# Autodesk Inventor assembly: Final AssemblyV6
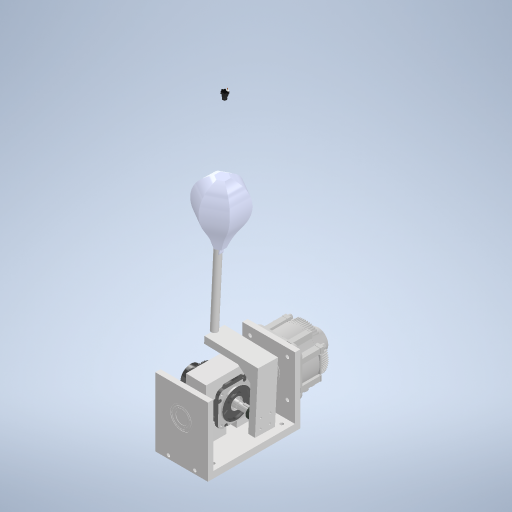
[picture p0: Inventor's stored thumbnail of the model, 512x512]
Saved by Autodesk Inventor 2024 (Build 280153000, 153)
## iProperties
Created: 2024-03-22
Part Number: Final AssemblyV6
Document SubType Name: Assembly
Designer: yusuf
Author: yusuf
## Documents named in this file (16)
- C:\Users\yusuf\Documents\DodgeBot\design\hardware\CAD_FILES\Final AssemblyV6.iam
- C:\Users\yusuf\Documents\DodgeBot\design\hardware\CAD_FILES\FloorMount.ipt
- C:\Users\yusuf\Documents\DodgeBot\design\hardware\CAD_FILES\145100992-9-skf_bearing_6209-2z_2\skf_bearing_6209-2z_2.iam
- C:\Users\yusuf\Documents\DodgeBot\design\hardware\CAD_FILES\FloorMountV2.ipt
- C:\Users\yusuf\Documents\DodgeBot\design\hardware\CAD_FILES\FloorMountFacePlate.ipt
- C:\Users\yusuf\Documents\DodgeBot\design\hardware\CAD_FILES\YASKAWA_USA_SGM7G30A6A61\AIS2024\SGM7G-30A6A61.iam
- C:\Users\yusuf\Documents\DodgeBot\design\hardware\CAD_FILES\grainger-big\grainger-big.iam
- C:\Users\yusuf\Documents\DodgeBot\design\hardware\CAD_FILES\FrontPlatePostNoKey.ipt
- C:\Users\yusuf\Documents\DodgeBot\design\hardware\CAD_FILES\EndEffector.ipt
- C:\Users\yusuf\Documents\DodgeBot\design\hardware\CAD_FILES\Speedbag\Speedbag.ipt
- C:\Users\yusuf\Documents\DodgeBot\design\hardware\CAD_FILES\grainger-small\grainger-small.iam
- C:\Users\yusuf\Documents\DodgeBot\design\hardware\CAD_FILES\SGM7G_20AxA61\SGM7G-20xxA61\ProE\SGM7G-20__a61_ProE\ProE\sgm7g_20__a61\sgm7g_20__a61.iam
- C:\Users\yusuf\Documents\DodgeBot\design\hardware\CAD_FILES\Post.ipt
- C:\Users\yusuf\Documents\DodgeBot\design\hardware\CAD_FILES\FrontPlatePostEndSide.ipt
- C:\Users\yusuf\Documents\DodgeBot\design\hardware\CAD_FILES\FrontPlateV3.ipt
- C:\Users\yusuf\Documents\DodgeBot\design\hardware\CAD_FILES\1000TVL v6\1000TVL v6.ipt
## Components (16 placed, 15 different names)
1. FloorMountV2:1 — Rigid:1, Rigid:2
2. FloorMountFacePlate:2 — Rigid:1, Rotational:1
3. skf_bearing_6209-2z_2:1 [sub-assembly] — Rotational:1, Rotational:10
4. skf_bearing_6209-2z_2:2 [sub-assembly] — Rotational:2
5. SGM7G-30A6A61:1 [sub-assembly] — Rigid:3, Rigid:10
6. FloorMount:1 — Rigid:2, Rotational:2, Rigid:3
7. grainger-big:1 [sub-assembly] — Rigid:10
8. EndEffector:1 — Rigid:7, Rotational:16, Rigid:15
9. Speedbag:1 — Rigid:6
10. grainger-small:1 [sub-assembly] — Rigid:12, Rotational:16
11. sgm7g_20__a61:1 [sub-assembly] — Rigid:12, Rotational:11
12. Post:1 — Rigid:6, Rigid:7
13. FrontPlatePostEndSide:1 — Rotational:10, Rigid:13
14. FrontPlateV3:1 — Rigid:13, Rotational:11, Rigid:14
15. FrontPlatePostNoKey:1 — Rigid:14
16. 1000TVL v6:1 — Rigid:15
## Relationships (15: WeldJoint 10, RevoluteJoint 5)
- Rigid:1 [WeldJoint]: FloorMountV2:1 ↔ FloorMountFacePlate:2
- Rotational:1 [RevoluteJoint]: FloorMountFacePlate:2 ↔ skf_bearing_6209-2z_2:1
- Rigid:2 [WeldJoint]: FloorMountV2:1 ↔ FloorMount:1
- Rotational:2 [RevoluteJoint]: skf_bearing_6209-2z_2:2 ↔ FloorMount:1
- Rigid:3 [WeldJoint]: SGM7G-30A6A61:1 ↔ FloorMount:1
- Rigid:10 [WeldJoint] (-31.623 mm): SGM7G-30A6A61:1 ↔ grainger-big:1
- Rigid:6 [WeldJoint]: Speedbag:1 ↔ Post:1
- Rigid:7 [WeldJoint]: EndEffector:1 ↔ Post:1
- Rigid:12 [WeldJoint]: grainger-small:1 ↔ sgm7g_20__a61:1
- Rotational:10 [RevoluteJoint]: skf_bearing_6209-2z_2:1 ↔ FrontPlatePostEndSide:1
- Rigid:13 [WeldJoint]: FrontPlatePostEndSide:1 ↔ FrontPlateV3:1
- Rotational:11 [RevoluteJoint]: sgm7g_20__a61:1 ↔ FrontPlateV3:1
- Rigid:14 [WeldJoint]: FrontPlateV3:1 ↔ FrontPlatePostNoKey:1
- Rotational:16 [RevoluteJoint]: EndEffector:1 ↔ grainger-small:1
- Rigid:15 [WeldJoint] (762 mm): EndEffector:1 ↔ 1000TVL v6:1
